# Autodesk Inventor assembly: pandoras_box_R2
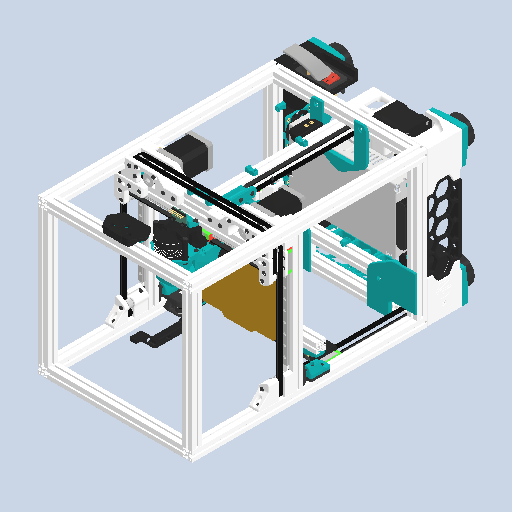
[picture p0: Inventor's stored thumbnail of the model, 512x512]
Saved by Autodesk Inventor 2026 (Build 300175050, 175E)
## iProperties
Created: 2023-04-16
Part Number: pandoras_box_R2
Document SubType Name: Assembly
Designer: tdxt
Sending System: Autodesk Translation Framework v12.4.0.73
Preprocessor: ST-DEVELOPER v19.2
Title: Pandora's Box v41.step
## Documents named in this file (9)
- D:\Github\Pandoras_Box\CAD\pandoras_box_R2\pandoras_box_R2\pandoras_box_R2.iam
- D:\Github\Pandoras_Box\CAD\pandoras_box_R2\pandoras_box_R2\Frame.iam
- D:\Github\Pandoras_Box\CAD\pandoras_box_R2\pandoras_box_R2\Gantry.iam
- D:\Github\Pandoras_Box\CAD\pandoras_box_R2\pandoras_box_R2\Z_Bed.iam
- D:\Github\Pandoras_Box\CAD\pandoras_box_R2\pandoras_box_R2\Electronics.iam
- D:\Github\Pandoras_Box\CAD\pandoras_box_R2\pandoras_box_R2\Skirts.iam
- D:\Github\Pandoras_Box\CAD\pandoras_box_R2\pandoras_box_R2\Spool_Holder.iam
- D:\Github\Pandoras_Box\CAD\pandoras_box_R2\pandoras_box_R2\Panels.iam
- D:\Github\Pandoras_Box\CAD\pandoras_box_R2\pandoras_box_R2\Multitool.ipt
## Components (8 placed, 8 different names)
1. Frame:1 [sub-assembly]
2. Gantry:1 [sub-assembly]
3. Z_Bed:1 [sub-assembly] — 表面齐平:1, 表面齐平:2, 表面齐平:3
4. Electronics:1 [sub-assembly]
5. Skirts:1 [sub-assembly] — 表面齐平:1, 表面齐平:2, 表面齐平:3
6. Spool_Holder:1 [sub-assembly]
7. Panels:1 [sub-assembly]
8. Multitool:1
## Relationships (3: Flush 3)
- 表面齐平:1 [Flush]: Z_Bed:1 ↔ Skirts:1
- 表面齐平:2 [Flush]: Z_Bed:1 ↔ Skirts:1
- 表面齐平:3 [Flush]: Z_Bed:1 ↔ Skirts:1
